# Autodesk Inventor assembly: Kinematic_DMD_ThorLabs_KM100
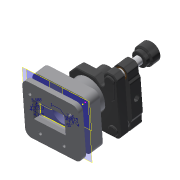
[picture p0: Inventor's stored thumbnail of the model, 180x180]
Saved by Autodesk Inventor 2019 (Build 230136000, 136)
## iProperties
Created: 2021-07-26
Part Number: Kinematic_DMD_ThorLabs_KM100
Document SubType Name: Assembly
Designer: wanghaoran
Author: wanghaoran
## Documents named in this file (4)
- C:\Users\wanghaoran\Dropbox\Promotion\SIMMO\Montage_STL\Kinematic_DMD_ThorLabs_KM100.iam
- C:\Users\wanghaoran\Dropbox\Promotion\SIMMO\Montage_STL\KM100-Solidworks.ipt
- C:\Users\wanghaoran\Dropbox\Promotion\SIMMO\Montage_STL\Cover_new.ipt
- C:\Users\wanghaoran\Dropbox\Promotion\SIMMO\Montage_STL\Adapter_DMD_KM100.ipt
## Components (3 placed, 3 different names)
1. KM100-Solidworks:1 — Mate:1, Mate:2, Angle:1
2. Cover_new:1 — Flush:1
3. Adapter_DMD_KM100:1 — Flush:1, Mate:1, Mate:2, Angle:1
## Relationships (4: Mate 2, Flush 1, Angle 1)
- Flush:1: Cover_new:1 ↔ Adapter_DMD_KM100:1
- Mate:1: KM100-Solidworks:1 ↔ Adapter_DMD_KM100:1
- Mate:2: KM100-Solidworks:1 ↔ Adapter_DMD_KM100:1
- Angle:1 (0 deg): KM100-Solidworks:1 ↔ Adapter_DMD_KM100:1
